# Autodesk Inventor assembly: SwitchOnTNutHolder
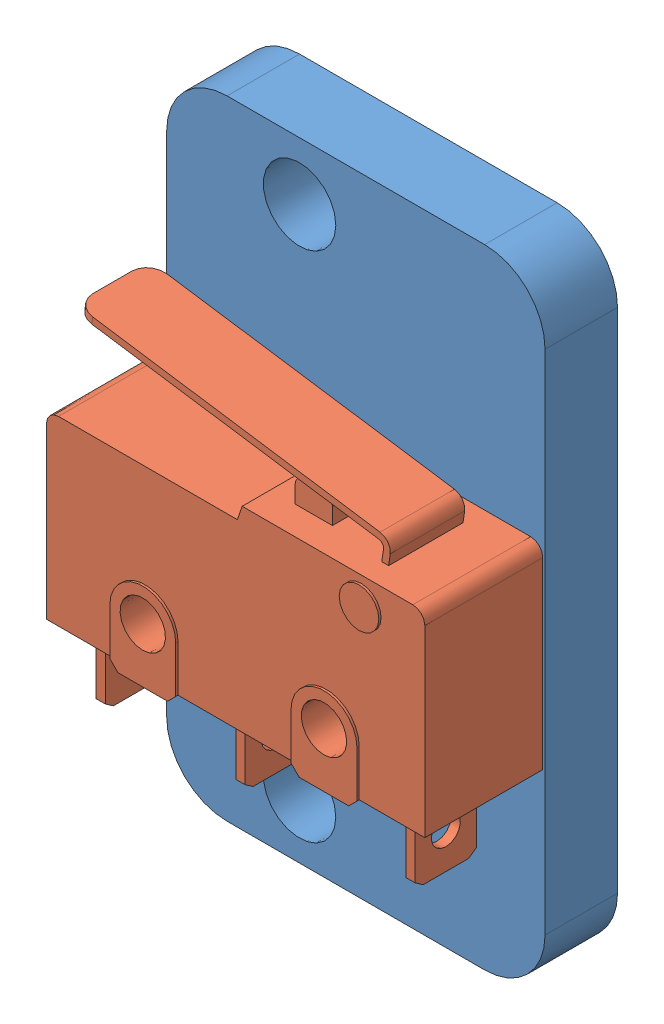
[picture p0: shaded view drawn from the shape stored in the file]
Saved by Autodesk Inventor 2018 (Build 220112000, 112)
## iProperties
Created: 2018-12-19
Part Number: SwitchOnTNutHolder
Document SubType Name: Assembly
Designer: ball
Author: ball
## Documents named in this file (3)
- C:\FTC\FTC8863CAD\2018Robot\SwitchOnTNutHolder.iam
- C:\FTC\FTC8863CAD\2018Robot\Switch on T nut holder.ipt
- C:\FTC\FTC8863CAD\Actobotics\605 parts\605630.ipt
## Components (2 placed, 2 different names)
1. Switch on T nut holder:1 — Mate:1, Mate:2, Mate:3
2. 605630:1 — Mate:1, Mate:2, Mate:3
## Relationships (3: Mate 3)
- Mate:1: Switch on T nut holder:1 ↔ 605630:1
- Mate:2: Switch on T nut holder:1 ↔ 605630:1
- Mate:3: Switch on T nut holder:1 ↔ 605630:1
